# Autodesk Inventor assembly: Finger_L1
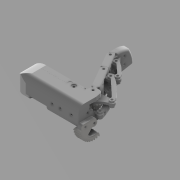
[picture p0: Inventor's stored thumbnail of the model, 180x180]
Saved by Autodesk Inventor 2016 (Build 200138000, 138)
## iProperties
Created: 2015-01-03
Part Number: Finger_L1
Document SubType Name: Assembly
Designer: 4ndreas
Mass: 91.442 g
Surface Area: 453.419 cm^2
Volume: 76.2212 cm^3
Density: 1.19969 g/cm^3
Author: 4ndreas
## Documents named in this file (16)
- C:\Users\4ndreas\Documents\Inventor\RobotARM v2\Gripper V1\Finger_L1.iam
- C:\Users\4ndreas\Documents\Inventor\RobotARM v2\Gripper V1\schnecke1.ipt
- C:\Users\4ndreas\Documents\Inventor\RobotARM v2\Gripper V1\DC-Motor_12V_60U-min1.ipt
- C:\Users\4ndreas\Documents\Inventor\RobotARM v2\Gripper V1\FingerPartA1.ipt
- C:\Users\4ndreas\Documents\Inventor\RobotARM v2\Gripper V1\FingerPartB1.ipt
- C:\Users\4ndreas\Documents\Inventor\RobotARM v2\Gripper V1\FingerTipp1.ipt
- C:\Users\4ndreas\Documents\Inventor\RobotARM v2\Gripper V1\Hebel_Basis1.ipt
- C:\Users\4ndreas\Documents\Inventor\RobotARM v2\Gripper V1\Hebel_Basis 21.ipt
- C:\Users\4ndreas\Documents\Inventor\RobotARM v2\Gripper V1\rotMount1.ipt
- C:\Users\4ndreas\Documents\Inventor\RobotARM v2\Gripper V1\kippGear.ipt
- C:\Users\4ndreas\Documents\Inventor\RobotARM v2\Gripper V1\deckel.ipt
- C:\Users\4ndreas\Documents\Inventor\RobotARM v2\Gripper V1\FingerTip_joint _v2_MIR.ipt
- C:\Users\4ndreas\Documents\Inventor\RobotARM v2\Gripper V1\3_hebenMount_2_dual1.ipt
- C:\Users\4ndreas\Documents\Inventor\RobotARM v2\Gripper V1\FingerTip_Mount dual1.ipt
- C:\Users\4ndreas\Documents\Inventor\RobotARM v2\Gripper V1\Hebel_B dual.ipt
- C:\Users\4ndreas\Documents\Inventor\RobotARM v2\Gripper V1\Hebel_dual.ipt
## Components (17 placed, 15 different names)
1. schnecke1:1 — Passend:4, Passend:19, Passend:21
2. DC-Motor_12V_60U-min1:1 — Passend:1, Winkel:2, Passend:21, Passend:22
3. FingerPartA1:1 — Fluchtend:1, Passend:9, Passend:8, Passend:14, Passend:17, Passend:15, Passend:19
4. FingerPartB1:1 — Fluchtend:1, Passend:9, Passend:8, Passend:11, Passend:10, Passend:25, Passend:27, Passend:28, Passend:29, Passend:30
5. FingerTipp1:1 — Passend:11, Passend:10, Fluchtend:3, Passend:26, Passend:31, Passend:36
6. Hebel_Basis1:1 — Passend:14, Passend:16, Passend:39
7. Hebel_Basis 21:1 — Passend:17, Passend:16, Passend:15, Passend:18, Passend:13, Passend:40
8. rotMount1:1 — Passend:19, Passend:18, Winkel:1, Passend:14, Passend:17, Passend:18, Passend:20, Winkel:2, Passend:22, Passend:23, Passend:24, Fluchtend:4
9. kippGear:1 — Passend:15, Passend:17, Passend:18
10. deckel:1 — Passend:23, Passend:24, Fluchtend:4
11. FingerTip_joint _v2_MIR:1 — Passend:25, Passend:26, Passend:32, Passend:35
12. 3_hebenMount_2_dual1:1 — Passend:28, Passend:29, Passend:34, Passend:37, Passend:41
13. FingerTip_Mount dual1:1 — Passend:27, Passend:30, Passend:33, Passend:38, Passend:42
14. Hebel_B dual:1 — Passend:31, Passend:33, Passend:36
15. Hebel_B dual:2 — Passend:32, Passend:34, Passend:35
16. Hebel_dual:1 — Passend:38, Passend:39, Passend:42
17. Hebel_dual:2 — Passend:37, Passend:40, Passend:41
## Relationships (48: Mate 42, Flush 4, Angle 2)
- Passend:4 [Mate]: schnecke1:1
- Passend:1 [Mate]: DC-Motor_12V_60U-min1:1
- Fluchtend:1 [Flush]: FingerPartA1:1 ↔ FingerPartB1:1
- Passend:9 [Mate]: FingerPartA1:1 ↔ FingerPartB1:1
- Passend:8 [Mate]: FingerPartA1:1 ↔ FingerPartB1:1
- Passend:11 [Mate]: FingerPartB1:1 ↔ FingerTipp1:1
- Passend:10 [Mate]: FingerPartB1:1 ↔ FingerTipp1:1
- Passend:14 [Mate]: FingerPartA1:1 ↔ Hebel_Basis1:1
- Passend:17 [Mate]: FingerPartA1:1 ↔ Hebel_Basis 21:1
- Passend:16 [Mate]: Hebel_Basis1:1 ↔ Hebel_Basis 21:1
- Passend:15 [Mate]: FingerPartA1:1 ↔ Hebel_Basis 21:1
- Passend:19 [Mate]: FingerPartA1:1 ↔ rotMount1:1
- Passend:18 [Mate]: Hebel_Basis 21:1 ↔ rotMount1:1
- Passend:13 [Mate]: Hebel_Basis 21:1
- Winkel:1 [Angle] (90 deg): rotMount1:1
- Fluchtend:2 [Flush] (36.5 mm)
- Fluchtend:3 [Flush]: FingerTipp1:1
- Passend:14 [Mate]: rotMount1:1
- Passend:15 [Mate]: kippGear:1
- Passend:16 [Mate]
- Passend:17 [Mate]: rotMount1:1 ↔ kippGear:1
- Passend:18 [Mate]: rotMount1:1 ↔ kippGear:1
- Passend:19 [Mate]: schnecke1:1
- Passend:20 [Mate]: rotMount1:1
- Winkel:2 [Angle] (0 deg): DC-Motor_12V_60U-min1:1 ↔ rotMount1:1
- Passend:21 [Mate] (2 mm): schnecke1:1 ↔ DC-Motor_12V_60U-min1:1
- Passend:22 [Mate]: DC-Motor_12V_60U-min1:1 ↔ rotMount1:1
- Passend:23 [Mate]: rotMount1:1 ↔ deckel:1
- Passend:24 [Mate]: rotMount1:1 ↔ deckel:1
- Fluchtend:4 [Flush]: rotMount1:1 ↔ deckel:1
- Passend:25 [Mate]: FingerPartB1:1 ↔ FingerTip_joint _v2_MIR:1
- Passend:26 [Mate]: FingerTipp1:1 ↔ FingerTip_joint _v2_MIR:1
- Passend:27 [Mate]: FingerPartB1:1 ↔ FingerTip_Mount dual1:1
- Passend:28 [Mate]: FingerPartB1:1 ↔ 3_hebenMount_2_dual1:1
- Passend:29 [Mate]: FingerPartB1:1 ↔ 3_hebenMount_2_dual1:1
- Passend:30 [Mate]: FingerPartB1:1 ↔ FingerTip_Mount dual1:1
- Passend:31 [Mate]: FingerTipp1:1 ↔ Hebel_B dual:1
- Passend:32 [Mate]: FingerTip_joint _v2_MIR:1 ↔ Hebel_B dual:2
- Passend:33 [Mate]: FingerTip_Mount dual1:1 ↔ Hebel_B dual:1
- Passend:34 [Mate]: 3_hebenMount_2_dual1:1 ↔ Hebel_B dual:2
- Passend:35 [Mate]: FingerTip_joint _v2_MIR:1 ↔ Hebel_B dual:2
- Passend:36 [Mate]: FingerTipp1:1 ↔ Hebel_B dual:1
- Passend:37 [Mate]: 3_hebenMount_2_dual1:1 ↔ Hebel_dual:2
- Passend:38 [Mate]: FingerTip_Mount dual1:1 ↔ Hebel_dual:1
- Passend:39 [Mate]: Hebel_Basis1:1 ↔ Hebel_dual:1
- Passend:40 [Mate]: Hebel_Basis 21:1 ↔ Hebel_dual:2
- Passend:41 [Mate]: 3_hebenMount_2_dual1:1 ↔ Hebel_dual:2
- Passend:42 [Mate]: FingerTip_Mount dual1:1 ↔ Hebel_dual:1
